# Autodesk Inventor assembly: Assembly_elevator
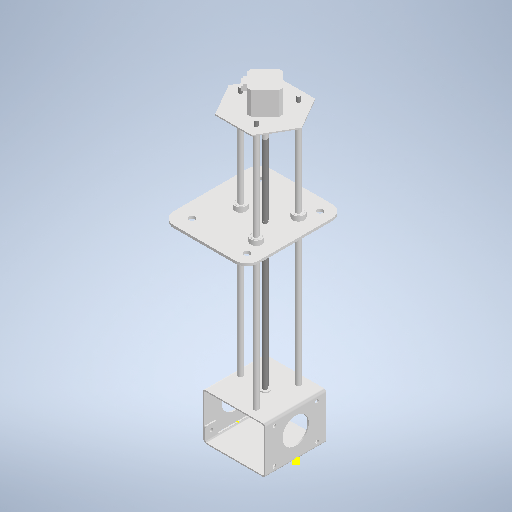
[picture p0: Inventor's stored thumbnail of the model, 512x512]
Saved by Autodesk Inventor 2025 (Build 290162010, 162A)
## iProperties
Created: 2025-03-04
Part Number: Assembly_elevator
Document SubType Name: Assembly
Designer: oskarjan
Author: oskarjan
## Documents named in this file (9)
- C:\Users\oskarjan\Documents\Kandidat_cad\Assembly_elevator.iam
- C:\Users\oskarjan\Documents\Kandidat_cad\Motorhållare4_gräsklippare.ipt
- C:\Users\oskarjan\Documents\10mm_rod.ipt
- C:\Users\oskarjan\Documents\Kandidat_cad\Motor_bracket_6mm_elevator.ipt
- C:\Users\oskarjan\Documents\Kandidat_cad\Nema17_42x42x38mm.ipt
- C:\Users\oskarjan\Documents\Kandidat_cad\linear_bearing_bushing_15x2x24.ipt
- C:\Users\oskarjan\Documents\Kandidat_cad\Linear_bearing_8x15x25mm.ipt
- C:\Users\oskarjan\Documents\Kandidat_cad\Elevator_baseplate_bracket2.ipt
- C:\Users\oskarjan\Documents\Kandidat_cad\Trappets_8mm.ipt
## Components (14 placed, 8 different names)
1. Motorhållare4_gräsklippare:1 — Mate:1, Mate:2, Mate:3, Mate:4, Mate:5, Mate:6, Mate:24, Mate:27
2. Nema17_42x42x38mm:1 — Mate:12, Mate:13, Mate:14
3. Elevator_baseplate_bracket2:1 — Mate:25, Mate:26, Mate:28, Mate:29
4. Trappets_8mm:1 — Mate:24, Mate:25, Mate:27
5. 10mm_rod:1 — Mate:4, Mate:5
6. 10mm_rod:2 — Mate:3, Mate:6, Mate:9, Mate:11
7. 10mm_rod:3 — Mate:1, Mate:2, Mate:10
8. Motor_bracket_6mm_elevator:1 — Mate:9, Mate:10, Mate:11, Mate:12, Mate:13, Mate:14
9. linear_bearing_bushing_15x2x24:1 — Mate:23, Flush:5, Mate:29
10. linear_bearing_bushing_15x2x24:2 — Mate:22, Flush:4, Mate:28
11. linear_bearing_bushing_15x2x24:3 — Mate:20, Mate:21, Mate:26
12. Linear_bearing_8x15x25mm:1 — Mate:23, Flush:5
13. Linear_bearing_8x15x25mm:2 — Mate:20, Mate:21
14. Linear_bearing_8x15x25mm:3 — Mate:22, Flush:4
## Relationships (24: Mate 22, Flush 2)
- Mate:1: Motorhållare4_gräsklippare:1 ↔ 10mm_rod:3
- Mate:2: Motorhållare4_gräsklippare:1 ↔ 10mm_rod:3
- Mate:3: Motorhållare4_gräsklippare:1 ↔ 10mm_rod:2
- Mate:4: Motorhållare4_gräsklippare:1 ↔ 10mm_rod:1
- Mate:5: Motorhållare4_gräsklippare:1 ↔ 10mm_rod:1
- Mate:6: Motorhållare4_gräsklippare:1 ↔ 10mm_rod:2
- Mate:9: 10mm_rod:2 ↔ Motor_bracket_6mm_elevator:1
- Mate:10: 10mm_rod:3 ↔ Motor_bracket_6mm_elevator:1
- Mate:11: 10mm_rod:2 ↔ Motor_bracket_6mm_elevator:1
- Mate:12: Nema17_42x42x38mm:1 ↔ Motor_bracket_6mm_elevator:1
- Mate:13: Nema17_42x42x38mm:1 ↔ Motor_bracket_6mm_elevator:1
- Mate:14: Nema17_42x42x38mm:1 ↔ Motor_bracket_6mm_elevator:1
- Mate:20: linear_bearing_bushing_15x2x24:3 ↔ Linear_bearing_8x15x25mm:2
- Mate:21: linear_bearing_bushing_15x2x24:3 ↔ Linear_bearing_8x15x25mm:2
- Mate:22: linear_bearing_bushing_15x2x24:2 ↔ Linear_bearing_8x15x25mm:3
- Flush:4: linear_bearing_bushing_15x2x24:2 ↔ Linear_bearing_8x15x25mm:3
- Mate:23: linear_bearing_bushing_15x2x24:1 ↔ Linear_bearing_8x15x25mm:1
- Flush:5: linear_bearing_bushing_15x2x24:1 ↔ Linear_bearing_8x15x25mm:1
- Mate:24: Motorhållare4_gräsklippare:1 ↔ Trappets_8mm:1
- Mate:25: Elevator_baseplate_bracket2:1 ↔ Trappets_8mm:1
- Mate:26: Elevator_baseplate_bracket2:1 ↔ linear_bearing_bushing_15x2x24:3
- Mate:27: Motorhållare4_gräsklippare:1 ↔ Trappets_8mm:1
- Mate:28: Elevator_baseplate_bracket2:1 ↔ linear_bearing_bushing_15x2x24:2
- Mate:29: Elevator_baseplate_bracket2:1 ↔ linear_bearing_bushing_15x2x24:1
